# Autodesk Inventor assembly: Leg
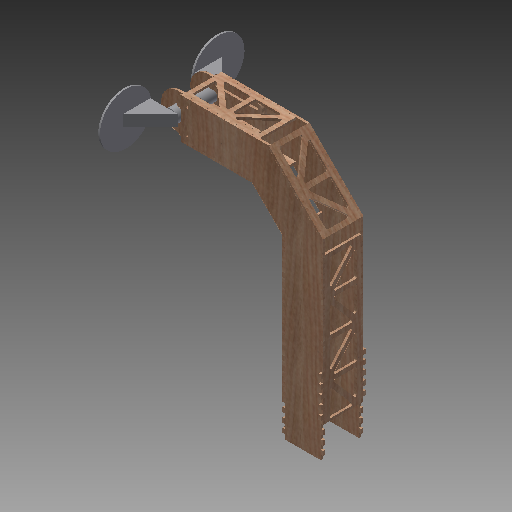
[picture p0: Inventor's stored thumbnail of the model, 512x512]
Saved by Autodesk Inventor 2019 (Build 230136000, 136)
## iProperties
Created: 2019-01-14
Part Number: Leg
Document SubType Name: Assembly
Designer: nxgam
Author: nxgam
## Documents named in this file (8)
- C:\Users\nxgam\Documents\CAD\Inventor\DiscoDraw\Leg.iam
- C:\Users\nxgam\Documents\CAD\Inventor\DiscoDraw\Leg.ipt
- C:\Users\nxgam\Documents\CAD\Inventor\DiscoDraw\CrossBar4.ipt
- C:\Users\nxgam\Documents\CAD\Inventor\DiscoDraw\CrossBar2.ipt
- C:\Users\nxgam\Documents\CAD\Inventor\DiscoDraw\CrossBar4Alt.ipt
- C:\Users\nxgam\Documents\CAD\Inventor\DiscoDraw\SuctionCup.ipt
- C:\Users\nxgam\Documents\CAD\Inventor\DiscoDraw\SuctionGrabberA.ipt
- C:\Users\nxgam\Documents\CAD\Inventor\DiscoDraw\SuctionGrabberB.ipt
## Components (12 placed, 7 different names)
1. Leg:1 — Flush:1, Flush:2, Flush:5, Flush:6, Mate:2, Flush:7, Flush:10, Mate:3, Mate:4, Mate:6
2. Leg:2 — Flush:1, Flush:2, Flush:3, Flush:4, Flush:11, Flush:12, Flush:13, Flush:14, Flush:16, Mate:5, Tangent:1, Mate:14
3. CrossBar4Alt:1 — Flush:15, Flush:16, Flush:17
4. CrossBar4:2 — Flush:13, Flush:14, Mate:4, Flush:15, Flush:17
5. CrossBar2:2 — Flush:6, Mate:2, Flush:7, Flush:8, Flush:9, Mate:9, Angle:1, Mate:14, Flush:22
6. CrossBar2:3 — Flush:8, Flush:9, Flush:10, Flush:22
7. CrossBar2:1 — Flush:3, Flush:4, Flush:5, Flush:11, Flush:12, Mate:3
8. SuctionCup:1 — Mate:10, Angle:1, Mate:11, Mate:12, Mate:13, Tangent:1
9. SuctionGrabberA:1 — Flush:20, Flush:21, Mate:7, Mate:10
10. SuctionGrabberA:2 — Flush:19, Flush:21, Mate:8, Mate:12
11. SuctionGrabberB:1 — Mate:5, Flush:18, Flush:20, Mate:7, Mate:11
12. SuctionGrabberB:2 — Mate:6, Flush:18, Flush:19, Mate:8, Mate:9, Mate:13
## Relationships (37: Flush 22, Mate 13, Angle 1, Tangent 1)
- Flush:1: Leg:1 ↔ Leg:2
- Flush:2: Leg:1 ↔ Leg:2
- Flush:3: Leg:2 ↔ CrossBar2:1
- Flush:4: Leg:2 ↔ CrossBar2:1
- Flush:5: Leg:1 ↔ CrossBar2:1
- Flush:6: Leg:1 ↔ CrossBar2:2
- Mate:2: Leg:1 ↔ CrossBar2:2
- Flush:7: Leg:1 ↔ CrossBar2:2
- Flush:8: CrossBar2:2 ↔ CrossBar2:3
- Flush:9: CrossBar2:2 ↔ CrossBar2:3
- Flush:10: Leg:1 ↔ CrossBar2:3
- Flush:11: Leg:2 ↔ CrossBar2:1
- Flush:12: Leg:2 ↔ CrossBar2:1
- Mate:3 (-5.08 mm): Leg:1 ↔ CrossBar2:1
- Flush:13: Leg:2 ↔ CrossBar4:2
- Flush:14: Leg:2 ↔ CrossBar4:2
- Mate:4: Leg:1 ↔ CrossBar4:2
- Flush:15: CrossBar4Alt:1 ↔ CrossBar4:2
- Flush:16: Leg:2 ↔ CrossBar4Alt:1
- Flush:17: CrossBar4Alt:1 ↔ CrossBar4:2
- Mate:5: Leg:2 ↔ SuctionGrabberB:1
- Mate:6: Leg:1 ↔ SuctionGrabberB:2
- Flush:18: SuctionGrabberB:1 ↔ SuctionGrabberB:2
- Flush:19: SuctionGrabberA:2 ↔ SuctionGrabberB:2
- Flush:20: SuctionGrabberA:1 ↔ SuctionGrabberB:1
- Flush:21: SuctionGrabberA:1 ↔ SuctionGrabberA:2
- Mate:7: SuctionGrabberA:1 ↔ SuctionGrabberB:1
- Mate:8: SuctionGrabberA:2 ↔ SuctionGrabberB:2
- Mate:9: CrossBar2:2 ↔ SuctionGrabberB:2
- Mate:10: SuctionCup:1 ↔ SuctionGrabberA:1
- Angle:1 (0 deg): CrossBar2:2 ↔ SuctionCup:1
- Mate:11: SuctionCup:1 ↔ SuctionGrabberB:1
- Mate:12: SuctionCup:1 ↔ SuctionGrabberA:2
- Mate:13: SuctionCup:1 ↔ SuctionGrabberB:2
- Tangent:1: Leg:2 ↔ SuctionCup:1
- Mate:14: Leg:2 ↔ CrossBar2:2
- Flush:22: CrossBar2:2 ↔ CrossBar2:3
